# Autodesk Inventor assembly: Respirador V3
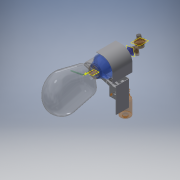
[picture p0: Inventor's stored thumbnail of the model, 180x180]
Saved by Autodesk Inventor 2019 (Build 230136000, 136)
## iProperties
Created: 2020-04-04
Part Number: Respirador V3
Document SubType Name: Assembly
Designer: Hermann
Author: Hermann
## Documents named in this file (12)
- E:\COVID19\Respirador V3\Respirador V3.iam
- E:\COVID19\Respirador V3\base.ipt
- E:\COVID19\Respirador V3\F006WMO310.ipt
- C:\Users\Hermann\Documents\Inventor\Content Center Files\R2019\en-US\BS 290 SKF(30)\BS 290 SKF - SKF 608.ipt
- E:\COVID19\Mask\Mancal.ipt
- E:\COVID19\Respirador V3\eixo.ipt
- E:\COVID19\Respirador V3\Haste.ipt
- C:\Users\Hermann\Documents\Inventor\Content Center Files\R2019\en-US\BS 290 SKF(30)\BS 290 SKF - SKF 6300.ipt
- E:\COVID19\Respirador V3\chapa.ipt
- E:\COVID19\Respirador V3\suporte ambu.ipt
- E:\COVID19\Respirador V3\Conjunto Ambu.iam
- E:\COVID19\Respirador V3\contato.ipt
## Components (14 placed, 11 different names)
1. base:1 — Mate:1, Mate:2, Mate:7, Mate:8, Mate:9, Flush:2, Flush:7
2. F006WMO310:1 — Mate:1, Mate:2
3. BS 290 SKF 608:1 — Mate:5, Mate:6, Mate:13, Mate:14
4. BS 290 SKF 608:3 — Mate:11, Mate:12, Mate:15
5. Mancal:1 — Mate:9, Flush:1, Mate:11, Mate:12
6. Mancal:2 — Mate:5, Mate:6, Mate:7, Mate:8, Flush:1, Flush:2, Mate:18
7. eixo:1 — Mate:13, Mate:14, Mate:15, Mate:16
8. Haste:1 — Mate:16, Flush:3, Flush:4, Mate:17, Mate:18, Mate:20, Flush:5, Flush:6
9. Haste:2 — Flush:3, Flush:4, Mate:17, Mate:19, Mate:21
10. BS 290 SKF 6300:1 — Mate:19, Mate:20
11. chapa:1 — Mate:21, Flush:5, Flush:6, Mate:23, Flush:8, Mate:24
12. suporte ambu:1 — Flush:7, Mate:22
13. Conjunto Ambu:1 [sub-assembly] — Mate:22
14. contato:1 — Mate:23, Flush:8, Mate:24
## Relationships (29: Mate 21, Flush 8)
- Mate:1: base:1 ↔ F006WMO310:1
- Mate:2: base:1 ↔ F006WMO310:1
- Mate:5: BS 290 SKF 608:1 ↔ Mancal:2
- Mate:6: BS 290 SKF 608:1 ↔ Mancal:2
- Mate:7: base:1 ↔ Mancal:2
- Mate:8 (5 mm): base:1 ↔ Mancal:2
- Mate:9: base:1 ↔ Mancal:1
- Flush:1: Mancal:1 ↔ Mancal:2
- Mate:11: BS 290 SKF 608:3 ↔ Mancal:1
- Mate:12: BS 290 SKF 608:3 ↔ Mancal:1
- Mate:13: BS 290 SKF 608:1 ↔ eixo:1
- Mate:14: BS 290 SKF 608:1 ↔ eixo:1
- Mate:15: BS 290 SKF 608:3 ↔ eixo:1
- Flush:2 (20 mm): base:1 ↔ Mancal:2
- Mate:16: eixo:1 ↔ Haste:1
- Flush:3: Haste:1 ↔ Haste:2
- Flush:4: Haste:1 ↔ Haste:2
- Mate:17 (12 mm): Haste:1 ↔ Haste:2
- Mate:18 (1 mm): Mancal:2 ↔ Haste:1
- Mate:19: Haste:2 ↔ BS 290 SKF 6300:1
- Mate:20: Haste:1 ↔ BS 290 SKF 6300:1
- Mate:21: Haste:2 ↔ chapa:1
- Flush:5 (20 mm): Haste:1 ↔ chapa:1
- Flush:6 (-40 mm): Haste:1 ↔ chapa:1
- Flush:7: base:1 ↔ suporte ambu:1
- Mate:22: suporte ambu:1 ↔ Conjunto Ambu:1
- Mate:23: chapa:1 ↔ contato:1
- Flush:8 (-10 mm): chapa:1 ↔ contato:1
- Mate:24 (15 mm): chapa:1 ↔ contato:1
